# Autodesk Inventor assembly: CaseRight
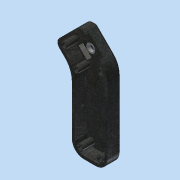
[picture p0: Inventor's stored thumbnail of the model, 180x180]
Saved by Autodesk Inventor 2015 (Build 190159000, 159)
## iProperties
Created: 2015-11-12
Part Number: CaseRight
Document SubType Name: Assembly
Designer: Raphael
Author: Raphael
## Documents named in this file (4)
- \\psf\Home\Documents\electric-skateboard\Remote\CAD\CaseRight.iam
- \\psf\Home\Documents\electric-skateboard\Remote\CAD\CaseRight.ipt
- \\psf\Home\Documents\electric-skateboard\Remote\CAD\Bearing.ipt
- \\psf\Home\Documents\electric-skateboard\Remote\CAD\MagnetSpring.ipt
## Components (3 placed, 3 different names)
1. CaseRight:1 — Mate:1, Mate:2, Mate:3, Mate:4, Mate:5
2. Bearing:1 — Mate:1, Mate:2
3. MagnetSpring:1 — Mate:3, Mate:4, Mate:5
## Relationships (5: Mate 5)
- Mate:1: CaseRight:1 ↔ Bearing:1
- Mate:2: CaseRight:1 ↔ Bearing:1
- Mate:3: CaseRight:1 ↔ MagnetSpring:1
- Mate:4: CaseRight:1 ↔ MagnetSpring:1
- Mate:5: CaseRight:1 ↔ MagnetSpring:1
